# Autodesk Inventor assembly: RelicArmLance
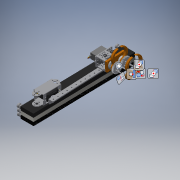
[picture p0: Inventor's stored thumbnail of the model, 180x180]
Saved by Autodesk Inventor 2017 (Build 210142000, 142)
## iProperties
Created: 2018-02-16
Part Number: RelicArmLance
Document SubType Name: Assembly
Designer: User
Author: User
## Documents named in this file (11)
- C:\Robotics\CAD\2017-18_CAD\RelicArmLance.iam
- C:\Robotics\CAD\2016-17_CAD\Lift2.iam
- C:\Robotics\CAD\COTSParts\Tetrix\39197_txm-485hb standard servo with horn.ipt
- C:\Robotics\CAD\COTSParts\Tetrix\ptp_tetrix_servoframe_bracket.ipt
- C:\Robotics\CAD\COTSParts\Tetrix\Tetrix angle 208mm.ipt
- C:\Robotics\CAD\COTSParts\Tetrix\Servo with servo blocks.ipt
- C:\Robotics\CAD\COTSParts\Tetrix\Tetrix Hub - axle.ipt
- C:\Robotics\CAD\2017-18_CAD\claw beta.ipt
- C:\Robotics\CAD\2017-18_CAD\claw attachment back.ipt
- C:\Robotics\CAD\COTSParts\Tetrix\Tetrix Gear 40T.ipt
- C:\Robotics\CAD\2016-17_CAD\Relic Arm Bar Space.ipt
## Components (17 placed, 10 different names)
1. Lift2:1 [sub-assembly] — Mate:4, Flush:1, Flush:2
2. 39197_txm-485hb standard servo with horn:1 — Mate:1, Mate:2, Mate:3, Flush:1, Mate:42, Mate:43, Mate:44
3. ptp_tetrix_servoframe_bracket:1 — Mate:1, Mate:2, Mate:3, Mate:4, Flush:2
4. Tetrix angle 208mm:1 — Mate:9, Mate:10, Angle:1, Mate:42, Mate:43, Mate:44
5. Servo with servo blocks:1 — Mate:9, Mate:10, Mate:19, Mate:20, Mate:21, Angle:1, Angle:2
6. Tetrix Hub - axle:1 — Mate:16, Mate:17, Mate:22, Mate:27
7. claw beta:1 — Mate:16, Mate:17, Mate:25, Mate:26, Mate:33, Flush:3
8. claw beta:2 — Mate:19, Mate:23, Mate:24, Mate:29, Flush:3
9. claw beta:3 — Mate:28, Mate:29, Mate:30, Tangent:1, Rotation:1
10. claw beta:4 — Mate:31, Mate:32, Mate:33, Tangent:2, Rotation:1
11. claw attachment back:1 — Mate:20, Mate:21, Mate:22, Mate:27, Angle:2
12. Tetrix Gear 40T:2 — Mate:23, Mate:24, Mate:28, Mate:30, Mate:34, Mate:35, Mate:36, Mate:37
13. Tetrix Gear 40T:3 — Mate:25, Mate:26, Mate:31, Mate:32, Mate:38, Mate:39, Mate:40, Mate:41
14. Relic Arm Bar Space:1 — Mate:34, Mate:35, Tangent:1
15. Relic Arm Bar Space:2 — Mate:36, Mate:37
16. Relic Arm Bar Space:3 — Mate:40, Mate:41
17. Relic Arm Bar Space:4 — Mate:38, Mate:39, Tangent:2
## Relationships (42: Mate 34, Flush 3, Tangent 2, Angle 2, RelateRotation 1)
- Mate:1: 39197_txm-485hb standard servo with horn:1 ↔ ptp_tetrix_servoframe_bracket:1
- Mate:2: 39197_txm-485hb standard servo with horn:1 ↔ ptp_tetrix_servoframe_bracket:1
- Mate:3: 39197_txm-485hb standard servo with horn:1 ↔ ptp_tetrix_servoframe_bracket:1
- Mate:4: Lift2:1 ↔ ptp_tetrix_servoframe_bracket:1
- Flush:1 (50.8 mm): Lift2:1 ↔ 39197_txm-485hb standard servo with horn:1
- Flush:2 (6.35 mm): Lift2:1 ↔ ptp_tetrix_servoframe_bracket:1
- Mate:9: Tetrix angle 208mm:1 ↔ Servo with servo blocks:1
- Mate:10: Tetrix angle 208mm:1 ↔ Servo with servo blocks:1
- Mate:16: Tetrix Hub - axle:1 ↔ claw beta:1
- Mate:17: Tetrix Hub - axle:1 ↔ claw beta:1
- Mate:19: Servo with servo blocks:1 ↔ claw beta:2
- Mate:20: Servo with servo blocks:1 ↔ claw attachment back:1
- Mate:21: Servo with servo blocks:1 ↔ claw attachment back:1
- Mate:22: Tetrix Hub - axle:1 ↔ claw attachment back:1
- Mate:23: claw beta:2 ↔ Tetrix Gear 40T:2
- Mate:24: claw beta:2 ↔ Tetrix Gear 40T:2
- Mate:25: claw beta:1 ↔ Tetrix Gear 40T:3
- Mate:26: claw beta:1 ↔ Tetrix Gear 40T:3
- Mate:27: Tetrix Hub - axle:1 ↔ claw attachment back:1
- Mate:28 (37.846 mm): claw beta:3 ↔ Tetrix Gear 40T:2
- Mate:29: claw beta:2 ↔ claw beta:3
- Mate:30: claw beta:3 ↔ Tetrix Gear 40T:2
- Mate:31 (37.846 mm): claw beta:4 ↔ Tetrix Gear 40T:3
- Mate:32: claw beta:4 ↔ Tetrix Gear 40T:3
- Mate:33: claw beta:1 ↔ claw beta:4
- Mate:34: Tetrix Gear 40T:2 ↔ Relic Arm Bar Space:1
- Mate:35: Tetrix Gear 40T:2 ↔ Relic Arm Bar Space:1
- Tangent:1: claw beta:3 ↔ Relic Arm Bar Space:1
- Mate:36: Tetrix Gear 40T:2 ↔ Relic Arm Bar Space:2
- Mate:37: Tetrix Gear 40T:2 ↔ Relic Arm Bar Space:2
- Mate:38: Tetrix Gear 40T:3 ↔ Relic Arm Bar Space:4
- Flush:3: claw beta:1 ↔ claw beta:2
- Mate:39: Tetrix Gear 40T:3 ↔ Relic Arm Bar Space:4
- Tangent:2: claw beta:4 ↔ Relic Arm Bar Space:4
- Mate:40: Tetrix Gear 40T:3 ↔ Relic Arm Bar Space:3
- Mate:41: Tetrix Gear 40T:3 ↔ Relic Arm Bar Space:3
- Angle:1 (0 deg): Tetrix angle 208mm:1 ↔ Servo with servo blocks:1
- Mate:42 (8.001 mm): 39197_txm-485hb standard servo with horn:1 ↔ Tetrix angle 208mm:1
- Mate:43 (8.001 mm): 39197_txm-485hb standard servo with horn:1 ↔ Tetrix angle 208mm:1
- Mate:44: 39197_txm-485hb standard servo with horn:1 ↔ Tetrix angle 208mm:1
- Angle:2 (270 deg): Servo with servo blocks:1 ↔ claw attachment back:1
- Rotation:1 [RelateRotation] (1 ul): claw beta:3 ↔ claw beta:4
